# Autodesk Inventor assembly: ASY TRM 050 shaft
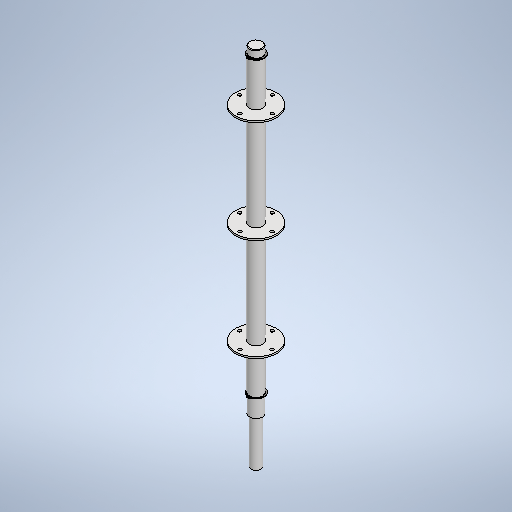
[picture p0: Inventor's stored thumbnail of the model, 512x512]
Saved by Autodesk Inventor 2025 (Build 290162010, 162A)
## iProperties
Created: 2024-09-11
Part Number: ASY TRM 050 shaft
Document SubType Name: Assembly
Designer: pokla
Author: pokla
## Documents named in this file (4)
- C:\Users\admin\YandexDisk-badmisterfox\домашниий пк\Inventor\BSH_Beshkino_bio_tank\ASY TRM 050 shaft.iam
- C:\Users\admin\YandexDisk-badmisterfox\домашниий пк\Inventor\BSH_Beshkino_bio_tank\TRM 028 main shaft.ipt
- C:\Users\admin\YandexDisk-badmisterfox\домашниий пк\Inventor\BSH_Beshkino_bio_tank\TRM 029 coupling ring.ipt
- C:\Users\admin\YandexDisk-badmisterfox\домашниий пк\Inventor\BSH_Beshkino_bio_tank\Content Center Files\en-US\CNS 9074(1)\CNS 9074 - 24 x 1,2(2).ipt
## Components (6 placed, 3 different names)
1. TRM 028 main shaft:1 — Rigid:2, Mate:1, Mate:2, Mate:3, Mate:4
2. TRM 029 coupling ring:1
3. TRM 029 coupling ring:2 — Rigid:2
4. TRM 029 coupling ring:3
5. CNS 9074 24 x 1,2:1 — Mate:1, Mate:2
6. CNS 9074 24 x 1,2:2 — Mate:3, Mate:4
## Relationships (7: Mate 4, WeldJoint 3)
- [WeldJoint] (-283.5 mm): TRM 028 main shaft:1 ↔ TRM 029 coupling ring:3
- Rigid:2 [WeldJoint] (-95 mm): TRM 028 main shaft:1 ↔ TRM 029 coupling ring:2
- [WeldJoint] (-472 mm): TRM 028 main shaft:1 ↔ TRM 029 coupling ring:1
- Mate:1: TRM 028 main shaft:1 ↔ CNS 9074 24 x 1,2:1
- Mate:2: TRM 028 main shaft:1 ↔ CNS 9074 24 x 1,2:1
- Mate:3: TRM 028 main shaft:1 ↔ CNS 9074 24 x 1,2:2
- Mate:4: TRM 028 main shaft:1 ↔ CNS 9074 24 x 1,2:2
